# Autodesk Inventor assembly: GI - 300
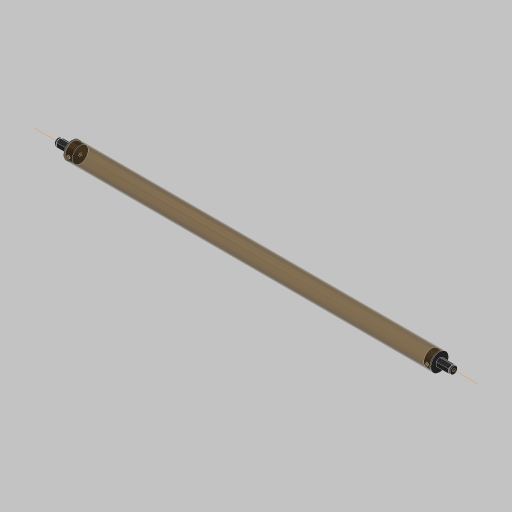
[picture p0: Inventor's stored thumbnail of the model, 512x512]
Saved by Autodesk Inventor 2023.5 (Build 275446000, 446)
## iProperties
Created: 2025-01-18
Part Number: GI - 300
Document SubType Name: Assembly
Designer: mavericks
Author: mavericks
## Documents named in this file (3)
- C:\Users\slick\OneDrive\Desktop\2025-ReefScape---CAD\ground intake\GI1\GI - 300.iam
- C:\Users\slick\OneDrive\Desktop\2025-ReefScape---CAD\ground intake\GI1\GI - 003.ipt
- C:\Users\slick\OneDrive\Desktop\2025-ReefScape---CAD\COMMON PARTS\WCP\WCP-0102.ipt
## Components (3 placed, 2 different names)
1. GI - 003:1 — Insert:1, Insert:2, Mate:3, Mate:4, Mate:5, Mate:6
2. WCP-0102:1 — Insert:1, Mate:4, Mate:5
3. WCP-0102:2 — Insert:2, Mate:3, Mate:6
## Relationships (6: Mate 4, Insert 2)
- Insert:1: GI - 003:1 ↔ WCP-0102:1
- Insert:2: GI - 003:1 ↔ WCP-0102:2
- Mate:3: GI - 003:1 ↔ WCP-0102:2
- Mate:4: GI - 003:1 ↔ WCP-0102:1
- Mate:5: GI - 003:1 ↔ WCP-0102:1
- Mate:6: GI - 003:1 ↔ WCP-0102:2
